# Autodesk Inventor assembly: XM430
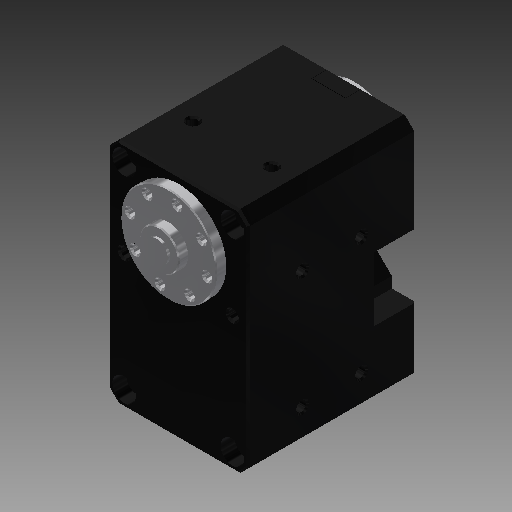
[picture p0: Inventor's stored thumbnail of the model, 512x512]
Saved by Autodesk Inventor 2023 (Build 270158000, 158)
## iProperties
Created: 2017-09-17
Part Number: XM430
Material: 一般
Document SubType Name: Assembly
Designer: TAKEMORI
Mass: 96.1801 g
Surface Area: 131.704 cm^2
Volume: 35.6223 cm^3
Density: 2.7 g/cm^3
Author: TAKEMORI
## Documents named in this file (4)
- C:\Users\michi\OneDrive - Kyoto University\lab\6_SHINOBI\FUHGA3\Design_Mechanism\Dynamixel\X430\XM430.iam
- C:\Users\michi\OneDrive - Kyoto University\lab\6_SHINOBI\FUHGA3\Design_Mechanism\Dynamixel\X430\DynamixelXM430_without_Hone.ipt
- C:\Users\michi\OneDrive - Kyoto University\lab\6_SHINOBI\FUHGA3\Design_Mechanism\Dynamixel\X430\DynamixelXM430_FreeHone.ipt
- C:\Users\michi\OneDrive - Kyoto University\lab\6_SHINOBI\FUHGA3\Design_Mechanism\Dynamixel\X430\DynamixelXM430_Hone.ipt
## Components (3 placed, 3 different names)
1. DynamixelXM430_without_Hone:1 — 挿入:1, 挿入:2, フラッシュ:1, フラッシュ:2, フラッシュ:3
2. DynamixelXM430_FreeHone:1 — 挿入:2
3. DynamixelXM430_Hone:1 — 挿入:1
## Relationships (5: Flush 3, Insert 2)
- 挿入:1 [Insert]: DynamixelXM430_without_Hone:1 ↔ DynamixelXM430_Hone:1
- 挿入:2 [Insert]: DynamixelXM430_without_Hone:1 ↔ DynamixelXM430_FreeHone:1
- フラッシュ:1 [Flush]: DynamixelXM430_without_Hone:1
- フラッシュ:2 [Flush]: DynamixelXM430_without_Hone:1
- フラッシュ:3 [Flush]: DynamixelXM430_without_Hone:1
